# Autodesk Inventor assembly: birdeye_rollUnit
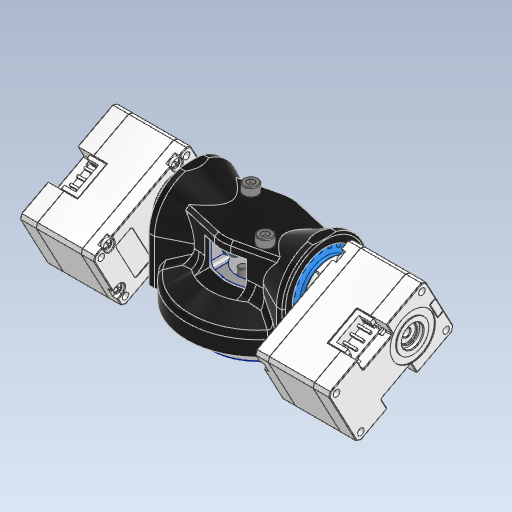
[picture p0: Inventor's stored thumbnail of the model, 512x512]
Saved by Autodesk Inventor 2024 (Build 280153000, 153)
## iProperties
Created: 2023-09-05
Part Number: birdeye_rollUnit
Document SubType Name: Assembly
Designer: michi
Mass: 77.7508 g
Surface Area: 466.75 cm^2
Volume: 48.4498 cm^3
Density: 1.60477 g/cm^3
Author: michi
## Documents named in this file (11)
- C:\Users\michi\OneDrive\default\robotis\DynamixelExamples\DynamixelXC330MiniArm\CAD_inventor\birdeye_shoulderUnit.iam
- C:\Users\michi\OneDrive - Kyoto University\lab\6_SHINOBI\FUHGA4\Design_Mechanism\05_birdeye\birdeye_shoulderUnit\birdeye_shoulderUnit_gear-large_under.ipt
- C:\Users\michi\OneDrive - Kyoto University\lab\6_SHINOBI\FUHGA4\Design_Mechanism\05_birdeye\birdeye_shoulderUnit\birdeye_shoulderUnit_actuator.iam
- C:\Users\michi\OneDrive - Kyoto University\lab\6_SHINOBI\FUHGA4\Design_Mechanism\05_birdeye\birdeye_shoulderUnit\_CRBT155A.iam
- C:\Users\michi\OneDrive - Kyoto University\lab\6_SHINOBI\FUHGA4\Design_Mechanism\05_birdeye\birdeye_shoulderUnit\_BA1730.iam
- C:\Users\michi\OneDrive - Kyoto University\lab\6_SHINOBI\FUHGA4\Design_Mechanism\05_birdeye\birdeye_shoulderUnit\birdeye_shoulderUnit_smallGearShaft.ipt
- C:\Users\michi\OneDrive - Kyoto University\lab\6_SHINOBI\FUHGA4\Design_Mechanism\05_birdeye\birdeye_shoulderUnit\birdeye_shoulderUnit_largeGearShaft.ipt
- C:\Users\michi\OneDrive - Kyoto University\lab\6_SHINOBI\FUHGA4\Design_Mechanism\05_birdeye\birdeye_shoulderUnit\birdeye_shoulderUnit_baseWasher.ipt
- C:\Users\michi\OneDrive - Kyoto University\lab\6_SHINOBI\FUHGA4\Design_Mechanism\05_birdeye\birdeye_shoulderUnit\birdeye_shoulderUnit_cover.ipt
- C:\Users\michi\OneDrive - Kyoto University\lab\6_SHINOBI\FUHGA4\Design_Mechanism\05_birdeye\birdeye__screw\Bolt_M2.5_6mm_CSH-ST-M2_5-6_203.ipt
- C:\Users\michi\OneDrive - Kyoto University\lab\6_SHINOBI\FUHGA4\Design_Mechanism\05_birdeye\birdeye_shoulderUnit\_LFF-0808.ipt
## Components (16 placed, 10 different names)
1. birdeye_shoulderUnit_gear-large_under:1
2. birdeye_shoulderUnit_actuator:1 [sub-assembly] — フラッシュ:1, リジッド:8
3. birdeye_shoulderUnit_actuator:2 [sub-assembly] — フラッシュ:1, リジッド:13
4. _CRBT155A:1 [sub-assembly] — メイト:2
5. _BA1730:1 [sub-assembly] — 回転:3
6. birdeye_shoulderUnit_smallGearShaft:1 — リジッド:8, メイト:10, メイト:11, メイト:16
7. birdeye_shoulderUnit_smallGearShaft:2 — リジッド:13, メイト:9, メイト:12, メイト:14
8. birdeye_shoulderUnit_largeGearShaft:1 — メイト:2, メイト:8, 回転:4, 回転:5, 回転:6, 回転:7, メイト:9, メイト:10, メイト:13, メイト:15
9. birdeye_shoulderUnit_baseWasher:1 — 回転:3, 回転:4, 回転:5, 回転:8, 回転:9
10. birdeye_shoulderUnit_cover:1 — 回転:6, 回転:7, 回転:10, 回転:11
11. Bolt_M2.5_6mm_CSH-ST-M2_5-6_203:1 — 回転:11
12. Bolt_M2.5_6mm_CSH-ST-M2_5-6_203:2 — 回転:10
13. Bolt_M2.5_6mm_CSH-ST-M2_5-6_203:3 — 回転:9
14. Bolt_M2.5_6mm_CSH-ST-M2_5-6_203:4 — 回転:8
15. _LFF-0808:1 — メイト:13, メイト:14, メイト:12
16. _LFF-0808:2 — メイト:15, メイト:16, メイト:11
## Relationships (24: Mate 11, RevoluteJoint 10, WeldJoint 2, Flush 1)
- [RevoluteJoint]: birdeye_shoulderUnit_gear-large_under:1 ↔ _CRBT155A:1
- メイト:2 [Mate]: _CRBT155A:1 ↔ birdeye_shoulderUnit_largeGearShaft:1
- [Mate]: _CRBT155A:1 ↔ birdeye_shoulderUnit_largeGearShaft:1
- フラッシュ:1 [Flush]: birdeye_shoulderUnit_actuator:1 ↔ birdeye_shoulderUnit_actuator:2
- メイト:8 [Mate]: birdeye_shoulderUnit_largeGearShaft:1
- 回転:3 [RevoluteJoint]: _BA1730:1 ↔ birdeye_shoulderUnit_baseWasher:1
- 回転:4 [RevoluteJoint]: birdeye_shoulderUnit_largeGearShaft:1 ↔ birdeye_shoulderUnit_baseWasher:1
- 回転:5 [RevoluteJoint]: birdeye_shoulderUnit_largeGearShaft:1 ↔ birdeye_shoulderUnit_baseWasher:1
- 回転:6 [RevoluteJoint]: birdeye_shoulderUnit_largeGearShaft:1 ↔ birdeye_shoulderUnit_cover:1
- 回転:7 [RevoluteJoint]: birdeye_shoulderUnit_largeGearShaft:1 ↔ birdeye_shoulderUnit_cover:1
- 回転:8 [RevoluteJoint]: birdeye_shoulderUnit_baseWasher:1 ↔ Bolt_M2.5_6mm_CSH-ST-M2_5-6_203:4
- 回転:9 [RevoluteJoint]: birdeye_shoulderUnit_baseWasher:1 ↔ Bolt_M2.5_6mm_CSH-ST-M2_5-6_203:3
- 回転:10 [RevoluteJoint]: birdeye_shoulderUnit_cover:1 ↔ Bolt_M2.5_6mm_CSH-ST-M2_5-6_203:2
- 回転:11 [RevoluteJoint]: birdeye_shoulderUnit_cover:1 ↔ Bolt_M2.5_6mm_CSH-ST-M2_5-6_203:1
- リジッド:8 [WeldJoint]: birdeye_shoulderUnit_actuator:1 ↔ birdeye_shoulderUnit_smallGearShaft:1
- リジッド:13 [WeldJoint]: birdeye_shoulderUnit_actuator:2 ↔ birdeye_shoulderUnit_smallGearShaft:2
- メイト:9 [Mate]: birdeye_shoulderUnit_smallGearShaft:2 ↔ birdeye_shoulderUnit_largeGearShaft:1
- メイト:10 [Mate]: birdeye_shoulderUnit_smallGearShaft:1 ↔ birdeye_shoulderUnit_largeGearShaft:1
- メイト:11 [Mate]: birdeye_shoulderUnit_smallGearShaft:1 ↔ _LFF-0808:2
- メイト:12 [Mate]: birdeye_shoulderUnit_smallGearShaft:2 ↔ _LFF-0808:1
- メイト:13 [Mate]: birdeye_shoulderUnit_largeGearShaft:1 ↔ _LFF-0808:1
- メイト:14 [Mate]: birdeye_shoulderUnit_smallGearShaft:2 ↔ _LFF-0808:1
- メイト:15 [Mate]: birdeye_shoulderUnit_largeGearShaft:1 ↔ _LFF-0808:2
- メイト:16 [Mate]: birdeye_shoulderUnit_smallGearShaft:1 ↔ _LFF-0808:2
